# Autodesk Inventor assembly: photodetector_assembly
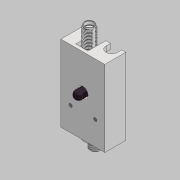
[picture p0: Inventor's stored thumbnail of the model, 180x180]
Saved by Autodesk Inventor 2021.4 (Build 254397000, 397)
## iProperties
Created: 2022-11-02
Part Number: photodetector_assembly
Document SubType Name: Assembly
Designer: Tilman Preuschoff
Author: Tilman Preuschoff
## Documents named in this file (7)
- C:\Users\Tilman Preuschoff\OneDrive\Dokumente\Elektronikprojekte\SFH2030_TIA\platine\small_version\case\assembly\photodetector_assembly.iam
- C:\Users\Tilman Preuschoff\OneDrive\Dokumente\Elektronikprojekte\SFH2030_TIA\platine\small_version\case\case.ipt
- C:\Users\Tilman Preuschoff\OneDrive\Dokumente\Elektronikprojekte\SFH2030_TIA\platine\small_version\case\assembly\SFH203_photodetector.iam
- C:\Users\Tilman Preuschoff\Documents\Inventor\Content Center Files\R2021\de-DE\DIN 84\DIN 84 - M2,5 x 5.ipt
- C:\Users\Tilman Preuschoff\Documents\Inventor\Content Center Files\R2021\de-DE\DIN 125-1  A\DIN 125 - A 6,4.ipt
- C:\Users\Tilman Preuschoff\Documents\Inventor\Content Center Files\R2021\de-DE\DIN 914\DIN 914 - M6 x 16.ipt
- C:\Users\Tilman Preuschoff\OneDrive\Dokumente\Elektronikprojekte\SFH2030_TIA\platine\small_version\case\cover.ipt
## Components (8 placed, 6 different names)
1. case:1 — Passend:1, Passend:3, Winkel:1, Passend:4, Winkel:2, Drehbar:4, Drehbar:5, Starr:1, Passend:5, Passend:7, Winkel:3, Passend:8
2. SFH203_photodetector:1 [sub-assembly] — Passend:4, Winkel:2, Drehbar:2, Drehbar:3, Drehbar:4, Passend:6
3. DIN 84 - ersetzt durch DIN EN ISO 1207 M2,5 x 5:3 — Drehbar:2
4. DIN 84 - ersetzt durch DIN EN ISO 1207 M2,5 x 5:4 — Drehbar:3
5. DIN 125-1 A A 6,4:1 — Starr:1
6. DIN 914 M6 x 16:1 — Drehbar:5
7. DIN 125-1 A A 6,4:2 — Passend:5, Passend:6
8. cover:1 — Passend:7, Winkel:3, Passend:8
## Relationships (15: Mate 7, RevoluteJoint 4, Angle 3, WeldJoint 1)
- Passend:1 [Mate]: case:1
- Passend:3 [Mate]: case:1
- Winkel:1 [Angle] (0 deg): case:1
- Passend:4 [Mate]: case:1 ↔ SFH203_photodetector:1
- Winkel:2 [Angle] (0 deg): case:1 ↔ SFH203_photodetector:1
- Drehbar:2 [RevoluteJoint]: SFH203_photodetector:1 ↔ DIN 84 - ersetzt durch DIN EN ISO 1207 M2,5 x 5:3
- Drehbar:3 [RevoluteJoint]: SFH203_photodetector:1 ↔ DIN 84 - ersetzt durch DIN EN ISO 1207 M2,5 x 5:4
- Drehbar:4 [RevoluteJoint]: case:1 ↔ SFH203_photodetector:1
- Drehbar:5 [RevoluteJoint] (6 mm): case:1 ↔ DIN 914 M6 x 16:1
- Starr:1 [WeldJoint]: case:1 ↔ DIN 125-1 A A 6,4:1
- Passend:5 [Mate]: case:1 ↔ DIN 125-1 A A 6,4:2
- Passend:6 [Mate]: SFH203_photodetector:1 ↔ DIN 125-1 A A 6,4:2
- Passend:7 [Mate]: case:1 ↔ cover:1
- Winkel:3 [Angle] (180 deg): case:1 ↔ cover:1
- Passend:8 [Mate]: case:1 ↔ cover:1
